# Autodesk Inventor assembly: 2.75 Omni AS, No Insert_MIR1
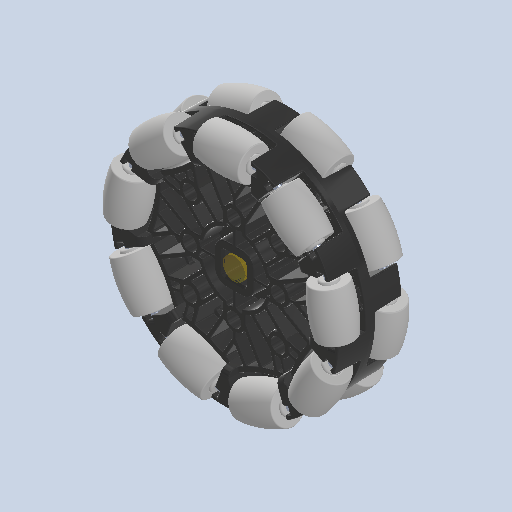
[picture p0: Inventor's stored thumbnail of the model, 512x512]
Saved by Autodesk Inventor 2023 (Build 270158000, 158)
## iProperties
Created: 2022-08-02
Part Number: 2.75 Omni AS, No Insert_MIR1
Document SubType Name: Assembly
Designer: Robodox
Author: ylu12
## Documents named in this file (2)
- C:\Users\Robodox\Documents\GitHub\2024-599Z\Cad\Library\VEX-CAD-Inventor-1.4.0\Motion\Wheels\Omni Wheel\2.75 Omni AS, No Insert_MIR1.iam
- C:\Users\Robodox\Documents\GitHub\2024-599Z\Cad\Library\VEX-CAD-Inventor-1.4.0\Motion\Wheels\Reference Files\2.75 Omni Antistatic_MIR1.ipt
## Components (1 placed, 1 different names)
1. 2.75 Omni Antistatic_MIR1:1 — Mate:8, Mate:7, Flush:4
## Relationships (3: Mate 2, Flush 1)
- Mate:8: 2.75 Omni Antistatic_MIR1:1
- Mate:7: 2.75 Omni Antistatic_MIR1:1
- Flush:4: 2.75 Omni Antistatic_MIR1:1
